# Autodesk Inventor assembly: car_2
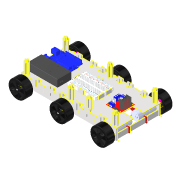
[picture p0: Inventor's stored thumbnail of the model, 180x180]
Saved by Autodesk Inventor 2022 (Build 260153000, 153)
## iProperties
Created: 2023-04-28
Part Number: car_2
Document SubType Name: Assembly
Designer: Johnny Jou
Author: Johnny Jou
## Documents named in this file (19)
- C:\Users\JOU\Desktop\git\Areo_Rider_Cabin\car\car_2.iam
- C:\Users\JOU\Desktop\git\Areo_Rider_Cabin\car\chassis_1_1_3.ipt
- C:\Users\JOU\Desktop\git\Areo_Rider_Cabin\car\外抓檔\25GA370.ipt
- C:\Users\JOU\Desktop\git\Areo_Rider_Cabin\car\chassis_1_5.ipt
- C:\Users\JOU\Desktop\git\Areo_Rider_Cabin\car\chassis_1_6.ipt
- C:\Users\JOU\Desktop\git\Areo_Rider_Cabin\car\plate_2.ipt
- C:\Users\JOU\Desktop\git\Areo_Rider_Cabin\car\bracket.ipt
- C:\Users\JOU\Desktop\git\Areo_Rider_Cabin\car\wheel.ipt
- C:\Users\JOU\Desktop\git\Areo_Rider_Cabin\car\chassis_1_7.ipt
- C:\Users\JOU\Desktop\git\Areo_Rider_Cabin\car\Coupling_0504.ipt
- C:\Users\JOU\Desktop\git\Areo_Rider_Cabin\car\2GT_36T.ipt
- C:\Users\JOU\Desktop\git\Areo_Rider_Cabin\car\axle 4_20.ipt
- C:\Users\JOU\Desktop\git\Areo_Rider_Cabin\car\bearing.ipt
- C:\Users\JOU\Desktop\git\Areo_Rider_Cabin\car\wheel_base_cover.ipt
- C:\Users\JOU\Desktop\git\Areo_Rider_Cabin\car\bracket_2.ipt
- C:\Users\JOU\Desktop\git\Areo_Rider_Cabin\car\外抓檔\BreadBoard.ipt
- C:\Users\JOU\Desktop\git\Areo_Rider_Cabin\car\外抓檔\arduino uno.ipt
- C:\Users\JOU\Desktop\git\Areo_Rider_Cabin\car\外抓檔\L298N.ipt
- C:\Users\JOU\Desktop\git\Areo_Rider_Cabin\car\外抓檔\電池和\3.7V 2X 18650 Battery Holder with On Off Switch_TOP.iam
## Components (72 placed, 18 different names)
1. 25GA370:1 — 貼合:7, 貼合:9, 貼合:183
2. 25GA370:2 — 貼合:7, 貼合:8, 貼合:49, 貼合:181
3. chassis_1_5:1 — 貼合:9, 齊平:5, 齊平:10, 齊平:11, 齊平:12, 齊平:13, 貼合:13, 貼合:14, 貼合:42, 貼合:43, 貼合:51
4. chassis_1_5:2 — 貼合:8, 齊平:5, 貼合:15, 貼合:16, 貼合:17, 貼合:18, 貼合:19, 貼合:20
5. chassis_1_6:1 — 齊平:7, 齊平:8, 齊平:9, 齊平:13, 貼合:13, 貼合:14
6. chassis_1_6:2 — 齊平:8, 齊平:10, 貼合:17, 貼合:18, 貼合:42, 貼合:43, 齊平:14, 貼合:44, 貼合:45, 齊平:15
7. chassis_1_6:3 — 齊平:9, 齊平:11, 貼合:19, 貼合:20
8. chassis_1_6:4 — 齊平:7, 齊平:12, 貼合:15, 貼合:16
9. plate_2:1 — 貼合:38, 貼合:40, 貼合:41, 貼合:50, 齊平:19, 貼合:116, 齊平:25, 貼合:185, 貼合:186, 貼合:187, 貼合:188, 貼合:189, 貼合:190, 貼合:191, 貼合:192, 貼合:193, 貼合:194, 貼合:195, 貼合:196, 貼合:197, 貼合:198, 貼合:199, 貼合:200, 貼合:203, 貼合:204, 貼合:205, 貼合:206, 貼合:207, 貼合:208, 貼合:209, 貼合:210, 貼合:211
10. chassis_1_1_3:1 — 齊平:14, 貼合:44, 貼合:45, 貼合:46, 貼合:47, 貼合:48, 貼合:49, 齊平:16, 貼合:108, 貼合:110, 貼合:111, 齊平:24, 貼合:171, 貼合:172, 貼合:182
11. chassis_1_1_3:2 — 齊平:15, 齊平:16, 貼合:50, 齊平:19, 貼合:52, 貼合:53, 貼合:54, 貼合:55, 貼合:56, 貼合:57, 貼合:109, 齊平:24, 齊平:25, 貼合:169, 貼合:170, 貼合:184
12. wheel:1 — 貼合:58, 貼合:59
13. chassis_1_7:1 — 貼合:51, 貼合:52, 貼合:53
14. chassis_1_7:2 — 貼合:54, 貼合:55, 貼合:56, 貼合:57
15. Coupling_0504:1 — 貼合:58, 貼合:59, 貼合:60, 貼合:61, 貼合:62, 貼合:63, 貼合:64, 貼合:66
16. 2GT_36T:1 — 貼合:60, 貼合:61, 貼合:62, 貼合:65
17. 2GT_36T:2 — 貼合:63, 貼合:64, 貼合:65, 貼合:70
18. axle 4_20:1 — 貼合:66, 貼合:69, 齊平:20
19. 軸承 GB/T 292-2007 類型 IN - 退回 B724 C:1 — 貼合:67, 貼合:68, 貼合:69, 齊平:20
20. wheel_base_cover:1 — 貼合:67, 貼合:68, 貼合:70, 貼合:171, 貼合:172
21. wheel:2
22. Coupling_0504:2
23. 2GT_36T:3
24. 2GT_36T:4
25. axle 4_20:2
26. 軸承 GB/T 292-2007 類型 IN - 退回 B724 C:2
27. wheel_base_cover:2 — 貼合:108, 貼合:109
28. wheel:3
29. Coupling_0504:4
30. 2GT_36T:7
31. 2GT_36T:8
32. axle 4_20:4
33. 軸承 GB/T 292-2007 類型 IN - 退回 B724 C:4
34. wheel_base_cover:4 — 貼合:110, 貼合:111
35. bracket:10 — 貼合:116, 貼合:210
36. bracket:9 — 貼合:211
37. wheel:4
38. Coupling_0504:5
39. 2GT_36T:9
40. 2GT_36T:10
41. axle 4_20:5
42. 軸承 GB/T 292-2007 類型 IN - 退回 B724 C:5
43. wheel_base_cover:5 — 貼合:169, 貼合:170
44. wheel:6
45. Coupling_0504:7 — 貼合:183
46. 2GT_36T:13
47. 2GT_36T:14 — 貼合:184
48. wheel:7
49. Coupling_0504:8 — 貼合:181
50. 2GT_36T:15
51. 2GT_36T:16 — 貼合:182
52. bracket_2:1 — 貼合:191, 貼合:196, 貼合:197
53. bracket_2:2 — 貼合:188, 貼合:192, 貼合:193
54. bracket_2:3 — 貼合:189, 貼合:194, 貼合:198, 貼合:202
55. bracket_2:4 — 貼合:190, 貼合:195, 貼合:199
56. bracket_2:5 — 貼合:185, 貼合:186, 貼合:187, 貼合:201
57. BreadBoard:1 — 貼合:200, 貼合:201, 貼合:202
58. L298N:1 — 貼合:203, 貼合:208, 貼合:209
59. arduino uno:1 — 貼合:204, 貼合:205, 貼合:206
60. 3.7V 2X 18650 Battery Holder with On Off Switch_TOP:1 [sub-assembly] — 貼合:207
61. bracket:7 — 貼合:38, 貼合:40
62. bracket:8 — 貼合:41
63. bracket:11
64. bracket:12
65. bracket:13
66. bracket:14
67. bracket:15
68. bracket:16
69. bracket:17
70. bracket:18
71. bracket:19
72. bracket:20
## Component patterns: (6 elements, first: bracket:7 + bracket:8)
## Relationships (162: Mate 144, Flush 18)
- 貼合:7 [Mate] (20 mm): 25GA370:1 ↔ 25GA370:2
- 貼合:8 [Mate]: 25GA370:2 ↔ chassis_1_5:2
- 貼合:9 [Mate]: 25GA370:1 ↔ chassis_1_5:1
- 齊平:5 [Flush]: chassis_1_5:1 ↔ chassis_1_5:2
- 齊平:7 [Flush]: chassis_1_6:1 ↔ chassis_1_6:4
- 齊平:8 [Flush]: chassis_1_6:1 ↔ chassis_1_6:2
- 齊平:9 [Flush]: chassis_1_6:1 ↔ chassis_1_6:3
- 齊平:10 [Flush]: chassis_1_5:1 ↔ chassis_1_6:2
- 齊平:11 [Flush]: chassis_1_5:1 ↔ chassis_1_6:3
- 齊平:12 [Flush]: chassis_1_5:1 ↔ chassis_1_6:4
- 齊平:13 [Flush]: chassis_1_5:1 ↔ chassis_1_6:1
- 貼合:13 [Mate]: chassis_1_5:1 ↔ chassis_1_6:1
- 貼合:14 [Mate]: chassis_1_5:1 ↔ chassis_1_6:1
- 貼合:15 [Mate]: chassis_1_5:2 ↔ chassis_1_6:4
- 貼合:16 [Mate]: chassis_1_5:2 ↔ chassis_1_6:4
- 貼合:17 [Mate]: chassis_1_5:2 ↔ chassis_1_6:2
- 貼合:18 [Mate]: chassis_1_5:2 ↔ chassis_1_6:2
- 貼合:19 [Mate]: chassis_1_5:2 ↔ chassis_1_6:3
- 貼合:20 [Mate]: chassis_1_5:2 ↔ chassis_1_6:3
- [Mate]: bracket:7 ↔ bracket:8
- [Mate]: bracket:7 ↔ bracket:8
- [Mate]: bracket:7 ↔ bracket:8
- 貼合:38 [Mate]: plate_2:1 ↔ bracket:7
- 貼合:40 [Mate]: plate_2:1 ↔ bracket:7
- 貼合:41 [Mate]: plate_2:1 ↔ bracket:8
- 貼合:42 [Mate]: chassis_1_5:1 ↔ chassis_1_6:2
- 貼合:43 [Mate]: chassis_1_5:1 ↔ chassis_1_6:2
- 齊平:14 [Flush]: chassis_1_6:2 ↔ chassis_1_1_3:1
- 貼合:44 [Mate]: chassis_1_6:2 ↔ chassis_1_1_3:1
- 貼合:45 [Mate]: chassis_1_6:2 ↔ chassis_1_1_3:1
- 貼合:46 [Mate]: chassis_1_1_3:1
- 貼合:47 [Mate]: chassis_1_1_3:1
- 貼合:48 [Mate]: chassis_1_1_3:1
- 貼合:49 [Mate]: 25GA370:2 ↔ chassis_1_1_3:1
- 齊平:15 [Flush]: chassis_1_6:2 ↔ chassis_1_1_3:2
- 齊平:16 [Flush]: chassis_1_1_3:1 ↔ chassis_1_1_3:2
- 貼合:50 [Mate]: plate_2:1 ↔ chassis_1_1_3:2
- 齊平:19 [Flush]: plate_2:1 ↔ chassis_1_1_3:2
- 貼合:51 [Mate]: chassis_1_5:1 ↔ chassis_1_7:1
- 貼合:52 [Mate]: chassis_1_1_3:2 ↔ chassis_1_7:1
- 貼合:53 [Mate]: chassis_1_1_3:2 ↔ chassis_1_7:1
- 貼合:54 [Mate]: chassis_1_1_3:2 ↔ chassis_1_7:2
- 貼合:55 [Mate]: chassis_1_1_3:2 ↔ chassis_1_7:2
- 貼合:56 [Mate]: chassis_1_1_3:2 ↔ chassis_1_7:2
- 貼合:57 [Mate]: chassis_1_1_3:2 ↔ chassis_1_7:2
- 貼合:58 [Mate]: wheel:1 ↔ Coupling_0504:1
- 貼合:59 [Mate]: wheel:1 ↔ Coupling_0504:1
- 貼合:60 [Mate]: Coupling_0504:1 ↔ 2GT_36T:1
- 貼合:61 [Mate]: Coupling_0504:1 ↔ 2GT_36T:1
- 貼合:62 [Mate]: Coupling_0504:1 ↔ 2GT_36T:1
- 貼合:63 [Mate]: Coupling_0504:1 ↔ 2GT_36T:2
- 貼合:64 [Mate]: Coupling_0504:1 ↔ 2GT_36T:2
- 貼合:65 [Mate]: 2GT_36T:1 ↔ 2GT_36T:2
- 貼合:66 [Mate]: Coupling_0504:1 ↔ axle 4_20:1
- 貼合:67 [Mate]: 軸承 GB/T 292-2007 類型 IN - 退回 B724 C:1 ↔ wheel_base_cover:1
- 貼合:68 [Mate]: 軸承 GB/T 292-2007 類型 IN - 退回 B724 C:1 ↔ wheel_base_cover:1
- 貼合:69 [Mate]: axle 4_20:1 ↔ 軸承 GB/T 292-2007 類型 IN - 退回 B724 C:1
- 齊平:20 [Flush]: axle 4_20:1 ↔ 軸承 GB/T 292-2007 類型 IN - 退回 B724 C:1
- 貼合:70 [Mate] (5 mm): 2GT_36T:2 ↔ wheel_base_cover:1
- [Mate]: wheel:2 ↔ Coupling_0504:2
- [Mate]: wheel:2 ↔ Coupling_0504:2
- [Mate]: Coupling_0504:2 ↔ 2GT_36T:3
- [Mate]: Coupling_0504:2 ↔ 2GT_36T:3
- [Mate]: Coupling_0504:2 ↔ 2GT_36T:3
- [Mate]: Coupling_0504:2 ↔ 2GT_36T:4
- [Mate]: Coupling_0504:2 ↔ 2GT_36T:4
- [Mate]: 2GT_36T:3 ↔ 2GT_36T:4
- [Mate]: Coupling_0504:2 ↔ axle 4_20:2
- [Mate]: 軸承 GB/T 292-2007 類型 IN - 退回 B724 C:2 ↔ wheel_base_cover:2
- [Mate]: 軸承 GB/T 292-2007 類型 IN - 退回 B724 C:2 ↔ wheel_base_cover:2
- [Mate]: axle 4_20:2 ↔ 軸承 GB/T 292-2007 類型 IN - 退回 B724 C:2
- [Flush]: axle 4_20:2 ↔ 軸承 GB/T 292-2007 類型 IN - 退回 B724 C:2
- [Mate] (5 mm): 2GT_36T:4 ↔ wheel_base_cover:2
- [Mate]: wheel:3 ↔ Coupling_0504:4
- [Mate]: wheel:3 ↔ Coupling_0504:4
- [Mate]: Coupling_0504:4 ↔ 2GT_36T:7
- [Mate]: Coupling_0504:4 ↔ 2GT_36T:7
- [Mate]: Coupling_0504:4 ↔ 2GT_36T:7
- [Mate]: Coupling_0504:4 ↔ 2GT_36T:8
- [Mate]: Coupling_0504:4 ↔ 2GT_36T:8
- [Mate]: 2GT_36T:7 ↔ 2GT_36T:8
- [Mate]: Coupling_0504:4 ↔ axle 4_20:4
- [Mate]: 軸承 GB/T 292-2007 類型 IN - 退回 B724 C:4 ↔ wheel_base_cover:4
- [Mate]: 軸承 GB/T 292-2007 類型 IN - 退回 B724 C:4 ↔ wheel_base_cover:4
- [Mate]: axle 4_20:4 ↔ 軸承 GB/T 292-2007 類型 IN - 退回 B724 C:4
- [Flush]: axle 4_20:4 ↔ 軸承 GB/T 292-2007 類型 IN - 退回 B724 C:4
- [Mate] (5 mm): 2GT_36T:8 ↔ wheel_base_cover:4
- 貼合:108 [Mate]: chassis_1_1_3:1 ↔ wheel_base_cover:2
- 貼合:109 [Mate]: chassis_1_1_3:2 ↔ wheel_base_cover:2
- 貼合:110 [Mate]: chassis_1_1_3:1 ↔ wheel_base_cover:4
- 貼合:111 [Mate]: chassis_1_1_3:1 ↔ wheel_base_cover:4
- [Mate]: bracket:10 ↔ bracket:9
- [Mate]: bracket:10 ↔ bracket:9
- [Mate]: bracket:10 ↔ bracket:9
- 貼合:116 [Mate]: plate_2:1 ↔ bracket:10
- 齊平:24 [Flush]: chassis_1_1_3:1 ↔ chassis_1_1_3:2
- 齊平:25 [Flush]: plate_2:1 ↔ chassis_1_1_3:2
- [Mate]: wheel:4 ↔ Coupling_0504:5
- [Mate]: wheel:4 ↔ Coupling_0504:5
- [Mate]: Coupling_0504:5 ↔ 2GT_36T:9
- [Mate]: Coupling_0504:5 ↔ 2GT_36T:9
- [Mate]: Coupling_0504:5 ↔ 2GT_36T:9
- [Mate]: Coupling_0504:5 ↔ 2GT_36T:10
- [Mate]: Coupling_0504:5 ↔ 2GT_36T:10
- [Mate]: 2GT_36T:9 ↔ 2GT_36T:10
- [Mate]: Coupling_0504:5 ↔ axle 4_20:5
- [Mate]: 軸承 GB/T 292-2007 類型 IN - 退回 B724 C:5 ↔ wheel_base_cover:5
- [Mate]: 軸承 GB/T 292-2007 類型 IN - 退回 B724 C:5 ↔ wheel_base_cover:5
- [Mate]: axle 4_20:5 ↔ 軸承 GB/T 292-2007 類型 IN - 退回 B724 C:5
- [Flush]: axle 4_20:5 ↔ 軸承 GB/T 292-2007 類型 IN - 退回 B724 C:5
- [Mate] (5 mm): 2GT_36T:10 ↔ wheel_base_cover:5
- [Mate]: wheel:6 ↔ Coupling_0504:7
- [Mate]: wheel:6 ↔ Coupling_0504:7
- [Mate]: Coupling_0504:7 ↔ 2GT_36T:13
- [Mate]: Coupling_0504:7 ↔ 2GT_36T:13
- [Mate]: Coupling_0504:7 ↔ 2GT_36T:13
- [Mate]: Coupling_0504:7 ↔ 2GT_36T:14
- [Mate]: Coupling_0504:7 ↔ 2GT_36T:14
- [Mate]: 2GT_36T:13 ↔ 2GT_36T:14
- 貼合:169 [Mate]: chassis_1_1_3:2 ↔ wheel_base_cover:5
- 貼合:170 [Mate]: chassis_1_1_3:2 ↔ wheel_base_cover:5
- 貼合:171 [Mate]: chassis_1_1_3:1 ↔ wheel_base_cover:1
- 貼合:172 [Mate]: chassis_1_1_3:1 ↔ wheel_base_cover:1
- [Mate]: wheel:7 ↔ Coupling_0504:8
- [Mate]: wheel:7 ↔ Coupling_0504:8
- [Mate]: Coupling_0504:8 ↔ 2GT_36T:15
- [Mate]: Coupling_0504:8 ↔ 2GT_36T:15
- [Mate]: Coupling_0504:8 ↔ 2GT_36T:15
- [Mate]: Coupling_0504:8 ↔ 2GT_36T:16
- [Mate]: Coupling_0504:8 ↔ 2GT_36T:16
- [Mate]: 2GT_36T:15 ↔ 2GT_36T:16
- 貼合:181 [Mate]: 25GA370:2 ↔ Coupling_0504:8
- 貼合:182 [Mate] (2 mm): chassis_1_1_3:1 ↔ 2GT_36T:16
- 貼合:183 [Mate]: 25GA370:1 ↔ Coupling_0504:7
- 貼合:184 [Mate] (2 mm): chassis_1_1_3:2 ↔ 2GT_36T:14
- 貼合:185 [Mate]: plate_2:1 ↔ bracket_2:5
- 貼合:186 [Mate]: plate_2:1 ↔ bracket_2:5
- 貼合:187 [Mate]: plate_2:1 ↔ bracket_2:5
- 貼合:188 [Mate]: plate_2:1 ↔ bracket_2:2
- 貼合:189 [Mate]: plate_2:1 ↔ bracket_2:3
- 貼合:190 [Mate]: plate_2:1 ↔ bracket_2:4
- 貼合:191 [Mate]: plate_2:1 ↔ bracket_2:1
- 貼合:192 [Mate]: plate_2:1 ↔ bracket_2:2
- 貼合:193 [Mate]: plate_2:1 ↔ bracket_2:2
- 貼合:194 [Mate]: plate_2:1 ↔ bracket_2:3
- 貼合:195 [Mate]: plate_2:1 ↔ bracket_2:4
- 貼合:196 [Mate]: plate_2:1 ↔ bracket_2:1
- 貼合:197 [Mate]: plate_2:1 ↔ bracket_2:1
- 貼合:198 [Mate]: plate_2:1 ↔ bracket_2:3
- 貼合:199 [Mate]: plate_2:1 ↔ bracket_2:4
- 貼合:200 [Mate]: plate_2:1 ↔ BreadBoard:1
- 貼合:201 [Mate]: bracket_2:5 ↔ BreadBoard:1
- 貼合:202 [Mate]: bracket_2:3 ↔ BreadBoard:1
- 貼合:203 [Mate]: plate_2:1 ↔ L298N:1
- 貼合:204 [Mate] (2 mm): plate_2:1 ↔ arduino uno:1
- 貼合:205 [Mate]: plate_2:1 ↔ arduino uno:1
- 貼合:206 [Mate]: plate_2:1 ↔ arduino uno:1
- 貼合:207 [Mate]: plate_2:1 ↔ 3.7V 2X 18650 Battery Holder with On Off Switch_TOP:1
- 貼合:208 [Mate]: plate_2:1 ↔ L298N:1
- 貼合:209 [Mate]: plate_2:1 ↔ L298N:1
- 貼合:210 [Mate]: plate_2:1 ↔ bracket:10
- 貼合:211 [Mate]: plate_2:1 ↔ bracket:9
## Named parameters: d54_d45 = 0 mm, d55_d46 = 0 mm, d56_d47 = 0 mm, d112_d98 = 0 mm, d113_d99 = 0 mm, d114_d100 = 0 mm, d115_d101 = 0 mm, d116_d102 = 0 mm, d117_d103 = 0 mm, d118_d104 = 0 mm, d119_d105 = 0 mm, d120_d106 = 0 mm, d121_d107 = 0 mm, d122_d108 = 0 mm, d123_d109 = 0 mm, d124_d110 = 0 mm, d125_d111 = 5 mm, d138_d98 = 0 mm, d139_d99 = 0 mm, d140_d100 = 0 mm, d141_d101 = 0 mm, d142_d102 = 0 mm, d143_d103 = 0 mm, d144_d104 = 0 mm, d145_d105 = 0 mm, d146_d106 = 0 mm, d147_d107 = 0 mm, d148_d108 = 0 mm, d149_d109 = 0 mm, d150_d110 = 0 mm, d151_d111 = 5 mm, d209_d54_d45 = 0 mm, d210_d55_d46 = 0 mm, d211_d56_d47 = 0 mm, d224_d98 = 0 mm, d225_d99 = 0 mm, d226_d100 = 0 mm, d227_d101 = 0 mm, d228_d102 = 0 mm, d229_d103 = 0 mm, d230_d104 = 0 mm, d231_d105 = 0 mm, d232_d106 = 0 mm, d233_d107 = 0 mm, d234_d108 = 0 mm, d235_d109 = 0 mm, d236_d110 = 0 mm, d237_d111 = 5 mm, d252_d98 = 0 mm, d253_d99 = 0 mm, d254_d100 = 0 mm, d255_d101 = 0 mm, d256_d102 = 0 mm, d257_d103 = 0 mm, d258_d104 = 0 mm, d259_d105 = 0 mm, d284_d252_d98 = 0 mm, d285_d253_d99 = 0 mm, d286_d254_d100 = 0 mm, d287_d255_d101 = 0 mm, d288_d256_d102 = 0 mm, d289_d257_d103 = 0 mm, d290_d258_d104 = 0 mm, d291_d259_d105 = 0 mm
